# Autodesk Inventor assembly: ASY MSC 100.1 roсket
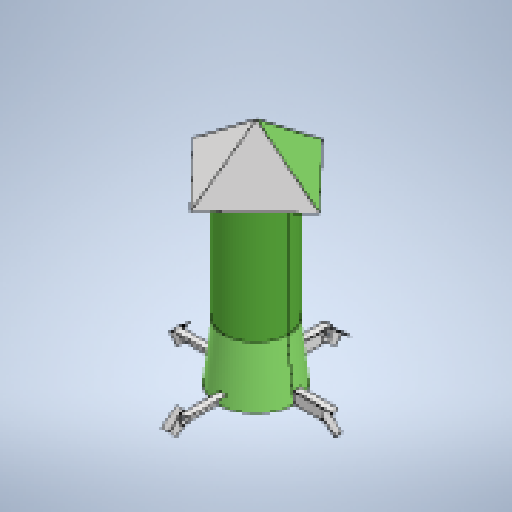
[picture p0: Inventor's stored thumbnail of the model, 512x512]
Saved by Autodesk Inventor 2025 (Build 290162010, 162A)
## iProperties
Created: 2024-05-19
Part Number: ASY MSC 100.1 roсket
Document SubType Name: Assembly
Designer: admin
Stock Number: ASY МОО 100.1 диффузор отбойник
Author: admin
## Documents named in this file (8)
- C:\Users\admin\YandexDisk-badmisterfox\домашниий пк\Inventor\Manturovo\Manturovo_Se-clar\ASY MSC 100.1 roсket.iam
- C:\Users\admin\YandexDisk-badmisterfox\домашниий пк\Inventor\Manturovo\Manturovo_Se-clar\MSC DIM 001 roсket sketch.ipt
- C:\Users\admin\YandexDisk-badmisterfox\домашниий пк\Inventor\Manturovo\Manturovo_Se-clar\MSC 101 roсket tail.ipt
- C:\Users\admin\YandexDisk-badmisterfox\домашниий пк\Inventor\Manturovo\Manturovo_Se-clar\MSC 102 roсket body.ipt
- C:\Users\admin\YandexDisk-badmisterfox\домашниий пк\Inventor\Manturovo\Manturovo_Se-clar\MSC 123 roсket pillar.ipt
- C:\Users\admin\YandexDisk-badmisterfox\домашниий пк\Inventor\Manturovo\Manturovo_Se-clar\MSC 124 roсket pillar.ipt
- C:\Users\admin\YandexDisk-badmisterfox\домашниий пк\Inventor\Manturovo\Manturovo_Se-clar\ASY MSC 100.3 roсket nose.iam
- C:\Users\admin\YandexDisk-badmisterfox\домашниий пк\Inventor\Manturovo\Manturovo_Se-clar\MSC 125 roсket pillar.ipt
## Components (16 placed, 7 different names)
1. MSC DIM 001 roсket sketch:1
2. MSC 101 roсket tail:1 — Rigid:1, Mate:2, Mate:3
3. MSC 102 roсket body:1 — Rigid:1, Flush:1, Mate:6
4. ASY MSC 100.3 roсket nose:1 [sub-assembly] — Flush:1, Mate:6, Angle:1
5. MSC 124 roсket pillar:1 — Rotational:1
6. MSC 123 roсket pillar:1 — Mate:3, Mate:4, Mate:5, Rotational:1
7. MSC 125 roсket pillar:1
8. MSC 124 roсket pillar:2
9. MSC 123 roсket pillar:2
10. MSC 125 roсket pillar:2
11. MSC 124 roсket pillar:3
12. MSC 123 roсket pillar:3
13. MSC 125 roсket pillar:3
14. MSC 124 roсket pillar:4
15. MSC 123 roсket pillar:4
16. MSC 125 roсket pillar:4
## Component patterns: (4 elements, first: MSC 124 roсket pillar:1 + MSC 123 roсket pillar:1 + MSC 125 roсket pillar:1)
## Relationships (9: Mate 5, WeldJoint 1, RevoluteJoint 1, Flush 1, Angle 1)
- Rigid:1 [WeldJoint]: MSC 101 roсket tail:1 ↔ MSC 102 roсket body:1
- Mate:2: MSC 101 roсket tail:1
- Mate:3: MSC 101 roсket tail:1 ↔ MSC 123 roсket pillar:1
- Mate:4: MSC 123 roсket pillar:1
- Mate:5 (100 mm): MSC 123 roсket pillar:1
- Rotational:1 [RevoluteJoint]: MSC 124 roсket pillar:1 ↔ MSC 123 roсket pillar:1
- Flush:1 (-30 mm): MSC 102 roсket body:1 ↔ ASY MSC 100.3 roсket nose:1
- Mate:6: MSC 102 roсket body:1 ↔ ASY MSC 100.3 roсket nose:1
- Angle:1 (0 deg): ASY MSC 100.3 roсket nose:1
